# Autodesk Inventor assembly: POM_T5_03
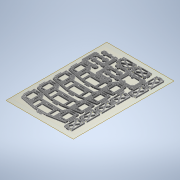
[picture p0: Inventor's stored thumbnail of the model, 180x180]
Saved by Autodesk Inventor 2022 (Build 260153000, 153)
## iProperties
Created: 2022-09-28
Part Number: POM_T5_03
Document SubType Name: Assembly
Designer: Masato
Author: Masato
## Documents named in this file (5)
- C:\Users\ヨコオリク\Documents\CITBrains\SUSTAINA-OP\Cam\POM_T5\POM_T5_03.iam
- C:\Users\ヨコオリク\Documents\CITBrains\SUSTAINA-OP\Cam\DisposableBoard.ipt
- C:\Users\ヨコオリク\Documents\CITBrains\SUSTAINA-OP\UpperBody\Head\Head_neck_diagonal.ipt
- C:\Users\ヨコオリク\Documents\CITBrains\SUSTAINA-OP\UpperBody\Trunk\Trunk_chest_frame.iam
- C:\Users\ヨコオリク\Documents\CITBrains\SUSTAINA-OP\UpperBody\Head\Head_camera_frame.ipt
## Components (18 placed, 4 different names)
1. DisposableBoard:1 — フラッシュ:1, フラッシュ:2, フラッシュ:3, フラッシュ:4, フラッシュ:9, フラッシュ:10, フラッシュ:12, フラッシュ:13
2. Head_camera_frame:8 — メイト:32, メイト:33, フラッシュ:13, メイト:35, メイト:36
3. Head_camera_frame:9 — メイト:34, メイト:35, メイト:36, メイト:42, メイト:44
4. Head_camera_frame:10 — メイト:40, メイト:41, メイト:42
5. Head_camera_frame:11 — メイト:39, メイト:43, メイト:48
6. Head_camera_frame:12 — メイト:46, メイト:47, メイト:48, メイト:49
7. Trunk_chest_frame:1 [sub-assembly] — メイト:6, フラッシュ:9, フラッシュ:10, メイト:24
8. Trunk_chest_frame:2 [sub-assembly]
9. Trunk_chest_frame:3 [sub-assembly]
10. Trunk_chest_frame:4 [sub-assembly] — メイト:33, メイト:41, メイト:47
11. Head_neck_diagonal:1 — メイト:17, メイト:19, フラッシュ:12, メイト:24
12. Head_neck_diagonal:2
13. Head_neck_diagonal:3
14. Head_neck_diagonal:4 — メイト:30
15. Head_neck_diagonal:5 — メイト:28, メイト:30, メイト:49
16. Head_neck_diagonal:6
17. Head_neck_diagonal:7 — メイト:31, メイト:43, メイト:44
18. Head_neck_diagonal:8
## Component patterns: (4 elements, first: Trunk_chest_frame:1), (4 elements, first: Head_neck_diagonal:1), (2 elements, first: Head_neck_diagonal:5), (2 elements, first: Head_neck_diagonal:7)
## Relationships (32: Mate 24, Flush 8)
- フラッシュ:1 [Flush]: DisposableBoard:1
- フラッシュ:2 [Flush]: DisposableBoard:1
- フラッシュ:3 [Flush]: DisposableBoard:1
- フラッシュ:4 [Flush]: DisposableBoard:1
- メイト:6 [Mate]: Trunk_chest_frame:1
- フラッシュ:9 [Flush] (-2 mm): DisposableBoard:1 ↔ Trunk_chest_frame:1
- フラッシュ:10 [Flush] (-2 mm): DisposableBoard:1 ↔ Trunk_chest_frame:1
- メイト:17 [Mate]: Head_neck_diagonal:1
- メイト:19 [Mate]: Head_neck_diagonal:1
- フラッシュ:12 [Flush] (2 mm): DisposableBoard:1 ↔ Head_neck_diagonal:1
- メイト:24 [Mate] (2.1 mm): Trunk_chest_frame:1 ↔ Head_neck_diagonal:1
- メイト:28 [Mate]: Head_neck_diagonal:5
- メイト:30 [Mate] (2.1 mm): Head_neck_diagonal:4 ↔ Head_neck_diagonal:5
- メイト:31 [Mate]: Head_neck_diagonal:7
- メイト:32 [Mate]: Head_camera_frame:8
- メイト:33 [Mate] (2.1 mm): Head_camera_frame:8 ↔ Trunk_chest_frame:4
- フラッシュ:13 [Flush] (2.1 mm): DisposableBoard:1 ↔ Head_camera_frame:8
- メイト:34 [Mate]: Head_camera_frame:9
- メイト:35 [Mate] (12 mm): Head_camera_frame:8 ↔ Head_camera_frame:9
- メイト:36 [Mate] (2.1 mm): Head_camera_frame:8 ↔ Head_camera_frame:9
- [Mate] (12 mm): Head_camera_frame:10 ↔ Head_camera_frame:11
- [Mate] (2.1 mm): Head_camera_frame:10 ↔ Head_camera_frame:11
- メイト:39 [Mate]: Head_camera_frame:11
- メイト:40 [Mate]: Head_camera_frame:10
- メイト:41 [Mate] (2.1 mm): Head_camera_frame:10 ↔ Trunk_chest_frame:4
- メイト:42 [Mate] (2.1 mm): Head_camera_frame:9 ↔ Head_camera_frame:10
- メイト:43 [Mate] (2.1 mm): Head_camera_frame:11 ↔ Head_neck_diagonal:7
- メイト:44 [Mate] (2.1 mm): Head_camera_frame:9 ↔ Head_neck_diagonal:7
- メイト:46 [Mate]: Head_camera_frame:12
- メイト:47 [Mate] (2.1 mm): Head_camera_frame:12 ↔ Trunk_chest_frame:4
- メイト:48 [Mate] (2.1 mm): Head_camera_frame:11 ↔ Head_camera_frame:12
- メイト:49 [Mate] (2.1 mm): Head_camera_frame:12 ↔ Head_neck_diagonal:5
## Named parameters: d136_d134 = 12 mm, d137_d135 = 2.1 mm
